# Autodesk Inventor assembly: Rear B2
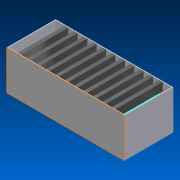
[picture p0: Inventor's stored thumbnail of the model, 180x180]
Saved by Autodesk Inventor 2012 (Build 160160000, 160)
## iProperties
Created: 2012-07-06
Part Number: Rear B2
Document SubType Name: Assembly
Designer: Hemant
Author: Hemant
## Documents named in this file (5)
- C:\Users\Hemant\Documents\Battery Boxes\BB REAR B\Rear B2.iam
- C:\Users\Hemant\Documents\Battery Boxes\BB REAR B\super large Battery Box Pastic 4.ipt
- C:\Users\Hemant\Documents\Battery Boxes\Batteries\CALB100AH final.ipt
- C:\Users\Hemant\Documents\Battery Boxes\BB REAR B\SPACER REAR B 1.ipt
- C:\Users\Hemant\Documents\Battery Boxes\BB REAR B\Spacer Rear 2.ipt
## Components (38 placed, 4 different names)
1. super large Battery Box Pastic 4:1 — Mate:2, Mate:3, Mate:4, Mate:6, Mate:7, Mate:8
2. SPACER REAR B 1:1 — Mate:5, Mate:6, Mate:7
3. SPACER REAR B 1:2
4. Spacer Rear 2:1 — Mate:8, Mate:9
5. Spacer Rear 2:2
6. Spacer Rear 2:3
7. Spacer Rear 2:4
8. Spacer Rear 2:5
9. Spacer Rear 2:6
10. Spacer Rear 2:7
11. Spacer Rear 2:8
12. Spacer Rear 2:9
13. Spacer Rear 2:10
14. Spacer Rear 2:11
15. CALB100AH final:1 — Mate:4
16. CALB100AH final:2 — Mate:2
17. CALB100AH final:3
18. CALB100AH final:4 — Mate:3
19. CALB100AH final:5
20. CALB100AH final:6
21. CALB100AH final:7
22. CALB100AH final:8 — Mate:5
23. CALB100AH final:9
24. CALB100AH final:10
25. CALB100AH final:11
26. CALB100AH final:12
27. CALB100AH final:13
28. CALB100AH final:14
29. CALB100AH final:15
30. CALB100AH final:16 — Mate:9
31. CALB100AH final:17
32. CALB100AH final:18
33. CALB100AH final:19
34. CALB100AH final:20
35. CALB100AH final:21
36. CALB100AH final:22
37. CALB100AH final:23
38. CALB100AH final:24
## Component patterns: (12 elements), (2 elements, first: SPACER REAR B 1:1), (11 elements, first: Spacer Rear 2:1), (2 elements, first: CALB100AH final:1), Component Pattern 1:2 (2 elements), Component Pattern 1:3 (2 elements), Component Pattern 1:4 (2 elements), Component Pattern 1:5 (2 elements), Component Pattern 1:6 (2 elements), Component Pattern 1:7 (2 elements), Component Pattern 1:8 (2 elements), Component Pattern 1:9 (2 elements), Component Pattern 1:10 (2 elements), Component Pattern 1:11 (2 elements), Component Pattern 1:12 (2 elements)
## Relationships (8: Mate 8)
- Mate:2: super large Battery Box Pastic 4:1 ↔ CALB100AH final:2
- Mate:3 (25.4 mm): super large Battery Box Pastic 4:1 ↔ CALB100AH final:4
- Mate:4 (15.24 mm): super large Battery Box Pastic 4:1 ↔ CALB100AH final:1
- Mate:5: SPACER REAR B 1:1 ↔ CALB100AH final:8
- Mate:6: super large Battery Box Pastic 4:1 ↔ SPACER REAR B 1:1
- Mate:7: super large Battery Box Pastic 4:1 ↔ SPACER REAR B 1:1
- Mate:8: super large Battery Box Pastic 4:1 ↔ Spacer Rear 2:1
- Mate:9: Spacer Rear 2:1 ↔ CALB100AH final:16
